# Autodesk Inventor assembly: table
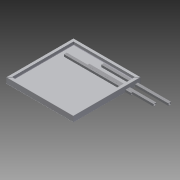
[picture p0: Inventor's stored thumbnail of the model, 180x180]
Saved by Autodesk Inventor 2013 (Build 170138000, 138)
## iProperties
Created: 2012-10-20
Part Number: table
Document SubType Name: Weldment
Designer: Istvan
Weld Material: Welded Aluminum-6061
Author: Istvan
## Documents named in this file (5)
- C:\Users\istvan.burbank\Documents\GitHub\Crown-Fire\CAD\Frame\Table\table.iam
- C:\Users\istvan.burbank\Documents\GitHub\Crown-Fire\CAD\Frame\Table\tableBottom.ipt
- C:\Users\istvan.burbank\Documents\GitHub\Crown-Fire\CAD\Frame\Table\tableSide.ipt
- C:\Users\istvan.burbank\Documents\GitHub\Crown-Fire\CAD\Templates\squareTube1.5x2.ipt
- C:\Users\istvan.burbank\Documents\GitHub\Crown-Fire\CAD\Frame\Table\slatHolder.ipt
## Components (8 placed, 3 different names)
1. tableBottom:1 — Mate:9, Mate:10, Mate:11, Mate:12, Mate:13, Mate:14
2. tableSide:1 — Mate:5, Mate:6, Flush:1, Mate:7, Mate:8, Mate:9
3. tableSide:2 — Mate:4, Mate:6, Flush:1, Flush:2, Mate:8, Mate:10
4. tableSide:3 — Mate:2, Mate:5, Flush:3, Mate:7
5. tableSide:4 — Mate:2, Mate:4, Flush:2, Flush:3, Mate:11
6. slatHolder:1 — Mate:14
7. slatHolder:2 — Mate:13
8. slatHolder:3 — Mate:12
## Relationships (15: Mate 12, Flush 3)
- Mate:2: tableSide:3 ↔ tableSide:4
- Mate:4: tableSide:2 ↔ tableSide:4
- Mate:5: tableSide:1 ↔ tableSide:3
- Mate:6: tableSide:1 ↔ tableSide:2
- Flush:1: tableSide:1 ↔ tableSide:2
- Flush:2: tableSide:2 ↔ tableSide:4
- Flush:3: tableSide:3 ↔ tableSide:4
- Mate:7: tableSide:1 ↔ tableSide:3
- Mate:8: tableSide:1 ↔ tableSide:2
- Mate:9: tableBottom:1 ↔ tableSide:1
- Mate:10: tableBottom:1 ↔ tableSide:2
- Mate:11: tableBottom:1 ↔ tableSide:4
- Mate:12: tableBottom:1 ↔ slatHolder:3
- Mate:13: tableBottom:1 ↔ slatHolder:2
- Mate:14: tableBottom:1 ↔ slatHolder:1
